# Autodesk Inventor assembly: sk8
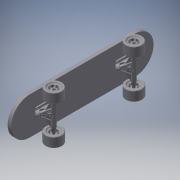
[picture p0: Inventor's stored thumbnail of the model, 180x180]
Saved by Autodesk Inventor 2017 SP1 (Build 210196100, 196)
## iProperties
Part Number: sk8
Material: 一般
Document SubType Name: Assembly
Designer: gisen
Author: gisen
## Documents named in this file (3)
- C:\Users\gisen\Documents\myElectricSk8\CAD\sk8.iam
- C:\Users\gisen\Documents\myElectricSk8\CAD\wheel_kit.iam
- C:\Users\gisen\Documents\myElectricSk8\CAD\board.ipt
## Components (3 placed, 2 different names)
1. wheel_kit:1 [sub-assembly] — フラッシュ:1, フラッシュ:2, メイト:1, フラッシュ:5, フラッシュ:6, メイト:2, 対称度:2
2. wheel_kit:2 [sub-assembly] — フラッシュ:1, フラッシュ:2, フラッシュ:3, フラッシュ:4, メイト:2, 対称度:2
3. board:1 — フラッシュ:3, フラッシュ:4, メイト:1, フラッシュ:6, メイト:5
## Relationships (11: Flush 6, Mate 4, Symmetry 1)
- フラッシュ:1 [Flush]: wheel_kit:1 ↔ wheel_kit:2
- フラッシュ:2 [Flush]: wheel_kit:1 ↔ wheel_kit:2
- フラッシュ:3 [Flush]: wheel_kit:2 ↔ board:1
- フラッシュ:4 [Flush]: wheel_kit:2 ↔ board:1
- メイト:1 [Mate]: wheel_kit:1 ↔ board:1
- フラッシュ:5 [Flush]: wheel_kit:1
- フラッシュ:6 [Flush]: wheel_kit:1 ↔ board:1
- メイト:2 [Mate] (450 mm): wheel_kit:1 ↔ wheel_kit:2
- 対称度:2 [Symmetry]: wheel_kit:1 ↔ wheel_kit:2
- メイト:4 [Mate]
- メイト:5 [Mate]: board:1
